# Autodesk Inventor assembly: FrameV3
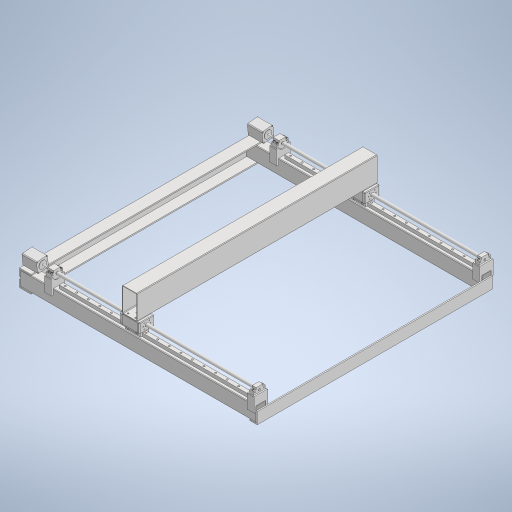
[picture p0: Inventor's stored thumbnail of the model, 512x512]
Saved by Autodesk Inventor 2023 (Build 270158000, 158)
## iProperties
Created: 2022-05-03
Part Number: FrameV3
Document SubType Name: Assembly
Designer: plebbb
Author: plebbb
## Documents named in this file (5)
- D:\Users\plebbb\Desktop\CNC_Project\FrameV3.iam
- D:\Users\plebbb\Desktop\CNC_Project\Ballscrew_Assembly.iam
- D:\Users\plebbb\Desktop\CNC_Project\X_GANTRY.iam
- D:\Users\plebbb\Desktop\CNC_Project\Steel_L_Bracket.ipt
- D:\Users\plebbb\Desktop\CNC_Project\5x3_Tube.ipt
## Components (8 placed, 4 different names)
1. Ballscrew_Assembly:1 [sub-assembly] — Mate:45, Mate:46
2. X_GANTRY:1 [sub-assembly] — Mate:30, Mate:31, Flush:4, Mate:32, Mate:33, Flush:5, Mate:38, Flush:9, Mate:40
3. X_GANTRY:2 [sub-assembly] — Mate:25, Mate:26, Mate:27, Mate:28, Mate:29, Mate:34, Mate:35, Mate:36, Mate:37, Flush:6, Flush:7, Mate:39, Flush:8
4. Ballscrew_Assembly:2 [sub-assembly] — Mate:25, Mate:26, Mate:27, Mate:28, Mate:29, Mate:43, Flush:11, Mate:44
5. Steel_L_Bracket:1 — Mate:30, Mate:31, Flush:4, Mate:34, Mate:37, Flush:6, Mate:41, Mate:42, Flush:10
6. Steel_L_Bracket:2 — Mate:32, Mate:33, Flush:5, Mate:35, Mate:36, Flush:7
7. Steel_L_Bracket:3 — Mate:38, Mate:39, Flush:8, Flush:9, Mate:40
8. 5x3_Tube:1 — Mate:43, Flush:11, Mate:44, Mate:45, Mate:46
## Relationships (38: Mate 28, Flush 10)
- [Mate]: Ballscrew_Assembly:1 ↔ X_GANTRY:1
- [Mate]: Ballscrew_Assembly:1 ↔ X_GANTRY:1
- [Flush]: Ballscrew_Assembly:1 ↔ X_GANTRY:1
- [Flush]: Ballscrew_Assembly:1 ↔ X_GANTRY:1
- [Mate]: Ballscrew_Assembly:1 ↔ X_GANTRY:1
- [Mate]: Ballscrew_Assembly:1 ↔ X_GANTRY:1
- [Mate]: Ballscrew_Assembly:1 ↔ X_GANTRY:1
- [Mate]: Ballscrew_Assembly:1 ↔ X_GANTRY:1
- Mate:25: X_GANTRY:2 ↔ Ballscrew_Assembly:2
- Mate:26: X_GANTRY:2 ↔ Ballscrew_Assembly:2
- Mate:27: X_GANTRY:2 ↔ Ballscrew_Assembly:2
- Mate:28: X_GANTRY:2 ↔ Ballscrew_Assembly:2
- Mate:29: X_GANTRY:2 ↔ Ballscrew_Assembly:2
- Mate:30: X_GANTRY:1 ↔ Steel_L_Bracket:1
- Mate:31: X_GANTRY:1 ↔ Steel_L_Bracket:1
- Flush:4: X_GANTRY:1 ↔ Steel_L_Bracket:1
- Mate:32: X_GANTRY:1 ↔ Steel_L_Bracket:2
- Mate:33: X_GANTRY:1 ↔ Steel_L_Bracket:2
- Flush:5: X_GANTRY:1 ↔ Steel_L_Bracket:2
- Mate:34: X_GANTRY:2 ↔ Steel_L_Bracket:1
- Mate:35: X_GANTRY:2 ↔ Steel_L_Bracket:2
- Mate:36: X_GANTRY:2 ↔ Steel_L_Bracket:2
- Mate:37: X_GANTRY:2 ↔ Steel_L_Bracket:1
- Flush:6: X_GANTRY:2 ↔ Steel_L_Bracket:1
- Flush:7: X_GANTRY:2 ↔ Steel_L_Bracket:2
- Mate:38: X_GANTRY:1 ↔ Steel_L_Bracket:3
- Mate:39: X_GANTRY:2 ↔ Steel_L_Bracket:3
- Flush:8: X_GANTRY:2 ↔ Steel_L_Bracket:3
- Flush:9: X_GANTRY:1 ↔ Steel_L_Bracket:3
- Mate:40: X_GANTRY:1 ↔ Steel_L_Bracket:3
- Mate:41: Steel_L_Bracket:1
- Mate:42: Steel_L_Bracket:1
- Flush:10: Steel_L_Bracket:1
- Mate:43: Ballscrew_Assembly:2 ↔ 5x3_Tube:1
- Flush:11: Ballscrew_Assembly:2 ↔ 5x3_Tube:1
- Mate:44: Ballscrew_Assembly:2 ↔ 5x3_Tube:1
- Mate:45: Ballscrew_Assembly:1 ↔ 5x3_Tube:1
- Mate:46: Ballscrew_Assembly:1 ↔ 5x3_Tube:1
